# Autodesk Inventor assembly: ASY Trommel
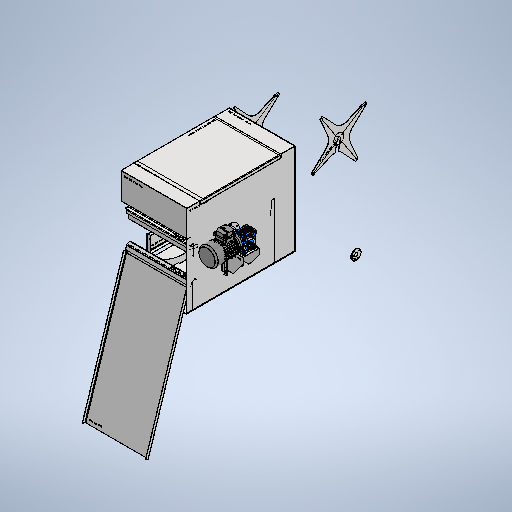
[picture p0: Inventor's stored thumbnail of the model, 512x512]
Saved by Autodesk Inventor 2025 (Build 290162010, 162A)
## iProperties
Created: 2024-08-07
Part Number: ASY Trommel
Document SubType Name: Assembly
Designer: pokla
Mass: 80063.4 g
Surface Area: 94462 cm^2
Volume: 14055.1 cm^3
Density: 5.6964 g/cm^3
Author: pokla
## Documents named in this file (29)
- C:\Users\admin\YandexDisk-badmisterfox\домашниий пк\Inventor\BSH_Beshkino_bio_tank\ASY Trommel.iam
- C:\Users\admin\YandexDisk-badmisterfox\домашниий пк\Inventor\BSH_Beshkino_bio_tank\TRM 011 bottom main.ipt
- C:\Users\admin\YandexDisk-badmisterfox\домашниий пк\Inventor\BSH_Beshkino_bio_tank\TRM 012 back main.ipt
- C:\Users\admin\YandexDisk-badmisterfox\домашниий пк\Inventor\BSH_Beshkino_bio_tank\TRM 013 top main.ipt
- C:\Users\admin\YandexDisk-badmisterfox\домашниий пк\Inventor\BSH_Beshkino_bio_tank\TRM 014 face main.ipt
- C:\Users\admin\YandexDisk-badmisterfox\домашниий пк\Inventor\BSH_Beshkino_bio_tank\TRM 015 left board main.ipt
- C:\Users\admin\YandexDisk-badmisterfox\домашниий пк\Inventor\BSH_Beshkino_bio_tank\TRM 017 sheet in.ipt
- C:\Users\admin\YandexDisk-badmisterfox\домашниий пк\Inventor\BSH_Beshkino_bio_tank\TRM 018 clipper.ipt
- C:\Users\admin\YandexDisk-badmisterfox\домашниий пк\Inventor\BSH_Beshkino_bio_tank\TRM 019 tray.ipt
- C:\Users\admin\YandexDisk-badmisterfox\домашниий пк\Inventor\BSH_Beshkino_bio_tank\TRM 021 bottom damper.ipt
- C:\Users\admin\YandexDisk-badmisterfox\домашниий пк\Inventor\BSH_Beshkino_bio_tank\TRM 022 back damper.ipt
- C:\Users\admin\YandexDisk-badmisterfox\домашниий пк\Inventor\BSH_Beshkino_bio_tank\TRM 023 face damper.ipt
- C:\Users\admin\YandexDisk-badmisterfox\домашниий пк\Inventor\BSH_Beshkino_bio_tank\TRM 024 top damper.ipt
- C:\Users\admin\YandexDisk-badmisterfox\домашниий пк\Inventor\BSH_Beshkino_bio_tank\TRM 025 left board damper.ipt
- C:\Users\admin\YandexDisk-badmisterfox\домашниий пк\Inventor\BSH_Beshkino_bio_tank\TRM 026 right board damper.ipt
- C:\Users\admin\YandexDisk-badmisterfox\домашниий пк\Inventor\BSH_Beshkino_bio_tank\TRM 027 tromel.ipt
- C:\Users\admin\YandexDisk-badmisterfox\домашниий пк\Inventor\BSH_Beshkino_bio_tank\TRM 028 main shaft.ipt
- C:\Users\admin\YandexDisk-badmisterfox\домашниий пк\Inventor\BSH_Beshkino_bio_tank\TRM 031 brush.ipt
- C:\Users\admin\YandexDisk-badmisterfox\домашниий пк\Inventor\BSH_Beshkino_bio_tank\ASY TRM 020 star.iam
- C:\Users\admin\YandexDisk-badmisterfox\домашниий пк\Inventor\BSH_Beshkino_bio_tank\ASY TRM 040 seal.iam
- C:\Users\admin\YandexDisk-badmisterfox\домашниий пк\Inventor\BSH_Beshkino_bio_tank\TRM 032 plate.ipt
- C:\Users\admin\YandexDisk-badmisterfox\домашниий пк\Inventor\BSH_Beshkino_bio_tank\TRM 029 coupling ring.ipt
- C:\Users\admin\YandexDisk-badmisterfox\домашниий пк\Inventor\BSH_Beshkino_bio_tank\TRM 016 right board main++.ipt
- C:\Users\admin\YandexDisk-badmisterfox\домашниий пк\Inventor\BSH_Beshkino_bio_tank\3d party\motor-reductor NMRV040\motor-reductor NMRV040.iam
- C:\Users\admin\YandexDisk-badmisterfox\домашниий пк\Inventor\BSH_Beshkino_bio_tank\TRM 034 motor pillar.ipt
- C:\Users\admin\YandexDisk-badmisterfox\домашниий пк\Inventor\BSH_Beshkino_bio_tank\TRM 035 motor pillar 2.ipt
- C:\Users\admin\YandexDisk-badmisterfox\домашниий пк\Inventor\BSH_Beshkino_bio_tank\TRM 036 box 1.ipt
- C:\Users\admin\YandexDisk-badmisterfox\домашниий пк\Inventor\BSH_Beshkino_bio_tank\TRM 037 box 2.ipt
- C:\Users\admin\YandexDisk-badmisterfox\домашниий пк\Inventor\BSH_Beshkino_bio_tank\TRM 038 facr wall.ipt
## Components (39 placed, 29 different names)
1. TRM 011 bottom main:1 — Rigid:25, Mate:11, Angle:3, Mate:23
2. TRM 012 back main:1 — Rigid:22, Mate:12
3. TRM 013 top main:1 — Mate:11, Mate:12, Rigid:33
4. TRM 014 face main:1 — Rigid:17
5. TRM 015 left board main:1 — Mate:2, Angle:1, Mate:5, Flush:1, Mate:7, Mate:8, Rigid:17, Rigid:24, Mate:10, Rigid:28, Angle:2, Mate:16, Mate:24
6. TRM 016 right board main++:1 — Rigid:29, Rigid:30, Rigid:32, Mate:20, Mate:21
7. TRM 017 sheet in:1 — Rigid:14, Angle:1, Rigid:22
8. TRM 018 clipper:1
9. TRM 019 tray:1 — Mate:13, Mate:14
10. TRM 021 bottom damper:1 — Rigid:28
11. TRM 022 back damper:1 — Rigid:24, Rigid:25, Rigid:29
12. TRM 023 face damper:1 — Mate:16, Rigid:34
13. TRM 024 top damper:1 — Flush:4, Mate:10, Tangent:1, Mate:13
14. TRM 026 right board damper:1 — Slider:1, Mate:17, Angle:3, Rigid:35, Rigid:36
15. TRM 028 main shaft:1 — Mate:1, Mate:2, Mate:4, Mate:15, Mate:17, Mate:18, Flush:5
16. TRM 027 tromel:1 — Rigid:14, Mate:4, Mate:5, Mate:9, Flush:4, Tangent:1
17. TRM 031 brush:1 — Flush:1, Rigid:21, Flush:3
18. TRM 029 coupling ring:1
19. ASY TRM 020 star:1 [sub-assembly] — Flush:3
20. ASY TRM 040 seal:1 [sub-assembly]
21. ASY TRM 040 seal:2 [sub-assembly] — Rigid:30
22. TRM 032 plate:1 — Rigid:21
23. TRM 021 bottom damper:2 — Rigid:32, Mate:19, Mate:22
24. TRM 025 left board damper:2 — Mate:19, Mate:22
25. TRM 013 top main:2 — Rigid:33
26. ASY TRM 020 star:2 [sub-assembly]
27. motor-reductor NMRV040:1 [sub-assembly] — Mate:15, Angle:2
28. 023 TRM face damper:2 — Slider:1, Rigid:34
29. TRM 029 coupling ring:2 — Mate:18, Flush:5
30. TRM 034 motor pillar:1 — Rigid:35
31. TRM 034 motor pillar:2 — Rigid:36, Rigid:37
32. TRM 035 motor pillar 2:1 — Rigid:37
33. ASY TRM 020 star:3 [sub-assembly]
34. TRM 036 box 1:1 — Rigid:38
35. TRM 037 box 2:1 — Mate:20, Mate:21, Rigid:38, Rigid:39
36. TRM 036 box 1:2 — Rigid:39
37. TRM 038 facr wall:1 — Mate:23, Mate:24
38. TRM 029 coupling ring:3
39. TRM 029 coupling ring:4
## Relationships (53: Mate 24, WeldJoint 19, Flush 5, Angle 3, Tangent 1, TranslationJoint 1)
- Rigid:14 [WeldJoint]: TRM 017 sheet in:1 ↔ TRM 027 tromel:1
- Mate:1: TRM 028 main shaft:1
- Mate:2: TRM 015 left board main:1 ↔ TRM 028 main shaft:1
- [Mate]: TRM 028 main shaft:1 ↔ TRM 029 coupling ring:1
- Mate:4: TRM 028 main shaft:1 ↔ TRM 027 tromel:1
- Angle:1 (0 deg): TRM 015 left board main:1 ↔ TRM 017 sheet in:1
- Mate:5: TRM 015 left board main:1 ↔ TRM 027 tromel:1
- Flush:1: TRM 015 left board main:1 ↔ TRM 031 brush:1
- [Mate]: TRM 031 brush:1 ↔ ASY TRM 020 star:1
- [Flush]: TRM 031 brush:1 ↔ ASY TRM 020 star:1
- Mate:7: TRM 015 left board main:1
- Mate:8: TRM 015 left board main:1
- Mate:9: TRM 027 tromel:1
- Rigid:17 [WeldJoint]: TRM 014 face main:1 ↔ TRM 015 left board main:1
- [WeldJoint]: TRM 015 left board main:1 ↔ ASY TRM 040 seal:1
- Rigid:21 [WeldJoint]: TRM 031 brush:1 ↔ TRM 032 plate:1
- Flush:3 (100 mm): TRM 031 brush:1 ↔ ASY TRM 020 star:1
- Rigid:22 [WeldJoint]: TRM 012 back main:1 ↔ TRM 017 sheet in:1
- [WeldJoint]: TRM 029 coupling ring:1 ↔ ASY TRM 020 star:1
- Rigid:24 [WeldJoint]: TRM 015 left board main:1 ↔ TRM 022 back damper:1
- Rigid:25 [WeldJoint]: TRM 011 bottom main:1 ↔ TRM 022 back damper:1
- Flush:4 (5 mm): TRM 024 top damper:1 ↔ TRM 027 tromel:1
- Mate:10: TRM 015 left board main:1 ↔ TRM 024 top damper:1
- Tangent:1: TRM 024 top damper:1 ↔ TRM 027 tromel:1
- Rigid:28 [WeldJoint]: TRM 015 left board main:1 ↔ TRM 021 bottom damper:1
- Rigid:29 [WeldJoint]: TRM 016 right board main++:1 ↔ TRM 022 back damper:1
- Rigid:30 [WeldJoint]: TRM 016 right board main++:1 ↔ ASY TRM 040 seal:2
- Rigid:32 [WeldJoint]: TRM 016 right board main++:1 ↔ TRM 021 bottom damper:2
- Mate:11: TRM 011 bottom main:1 ↔ TRM 013 top main:1
- Mate:12: TRM 012 back main:1 ↔ TRM 013 top main:1
- Mate:13: TRM 019 tray:1 ↔ TRM 024 top damper:1
- Mate:14: TRM 019 tray:1
- Rigid:33 [WeldJoint] (200 mm): TRM 013 top main:1 ↔ TRM 013 top main:2
- Mate:15: TRM 028 main shaft:1 ↔ motor-reductor NMRV040:1
- Angle:2 (0 deg): TRM 015 left board main:1 ↔ motor-reductor NMRV040:1
- Mate:16: TRM 015 left board main:1 ↔ TRM 023 face damper:1
- Slider:1 [TranslationJoint]: TRM 026 right board damper:1 ↔ 023 TRM face damper:2
- Mate:17: TRM 026 right board damper:1 ↔ TRM 028 main shaft:1
- Mate:18: TRM 028 main shaft:1 ↔ TRM 029 coupling ring:2
- Rigid:34 [WeldJoint] (120 mm): TRM 023 face damper:1 ↔ 023 TRM face damper:2
- Angle:3 (0 deg): TRM 011 bottom main:1 ↔ TRM 026 right board damper:1
- Rigid:35 [WeldJoint]: TRM 026 right board damper:1 ↔ TRM 034 motor pillar:1
- Rigid:36 [WeldJoint]: TRM 026 right board damper:1 ↔ TRM 034 motor pillar:2
- Rigid:37 [WeldJoint]: TRM 034 motor pillar:2 ↔ TRM 035 motor pillar 2:1
- Flush:5 (150 mm): TRM 028 main shaft:1 ↔ TRM 029 coupling ring:2
- Mate:19: TRM 021 bottom damper:2 ↔ TRM 025 left board damper:2
- Mate:20: TRM 016 right board main++:1 ↔ TRM 037 box 2:1
- Mate:21 (-2 mm): TRM 016 right board main++:1 ↔ TRM 037 box 2:1
- Rigid:38 [WeldJoint]: TRM 036 box 1:1 ↔ TRM 037 box 2:1
- Rigid:39 [WeldJoint]: TRM 037 box 2:1 ↔ TRM 036 box 1:2
- Mate:22: TRM 021 bottom damper:2 ↔ TRM 025 left board damper:2
- Mate:23: TRM 011 bottom main:1 ↔ TRM 038 facr wall:1
- Mate:24: TRM 015 left board main:1 ↔ TRM 038 facr wall:1
